# Autodesk Inventor assembly: Motor + Shaft
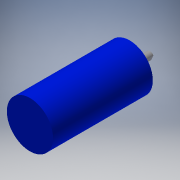
[picture p0: Inventor's stored thumbnail of the model, 180x180]
Saved by Autodesk Inventor 2016 (Build 200138000, 138)
## iProperties
Created: 2016-04-13
Part Number: Motor + Shaft
Document SubType Name: Assembly
Designer: schiu30
Author: schiu30
## Documents named in this file (3)
- C:\Users\Andrea\Documents\Dropbox\Capstone CAD\Motor + Attachment\Motor + Shaft.iam
- C:\Users\Andrea\Documents\Dropbox\Capstone CAD\Motor + Attachment\Motor Shaft.ipt
- C:\Users\Andrea\Documents\Dropbox\Capstone CAD\Motor + Attachment\Motor.ipt
## Components (2 placed, 2 different names)
1. Motor:1 — Flush:1, Flush:2, Flush:3, Mate:1, Mate:2
2. Motor Shaft:1 — Mate:1, Mate:2
## Relationships (5: Flush 3, Mate 2)
- Flush:1: Motor:1
- Flush:2: Motor:1
- Flush:3: Motor:1
- Mate:1: Motor:1 ↔ Motor Shaft:1
- Mate:2: Motor:1 ↔ Motor Shaft:1
